# Autodesk Inventor assembly: Custom Cover v0.3
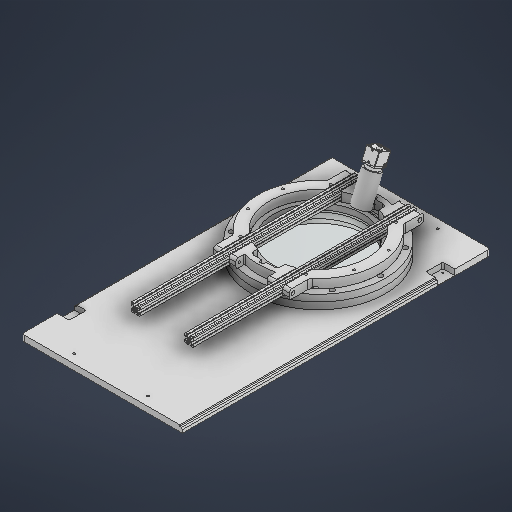
[picture p0: Inventor's stored thumbnail of the model, 512x512]
Saved by Autodesk Inventor 2025 (Build 290162000, 162)
## iProperties
Created: 2024-10-25
Part Number: Custom Cover v0.3
Document SubType Name: Assembly
Designer: mayhe
Author: mayhe
## Documents named in this file (15)
- C:\Users\mayhe\OneDrive\Documents\GitHub\In-situ-monitoring-of-powder-bed-fusion-additive-manufacturing\system_development\Orichalcum\v0.2\Hardware_design\custom-cover\Cover v 3\Custom Cover v0.3.iam
- C:\Users\mayhe\OneDrive\Documents\GitHub\In-situ-monitoring-of-powder-bed-fusion-additive-manufacturing\system_development\Orichalcum\v0.2\Hardware_design\custom-cover\cover\Updated Cover.ipt
- C:\Users\mayhe\OneDrive\Documents\GitHub\In-situ-monitoring-of-powder-bed-fusion-additive-manufacturing\system_development\Orichalcum\v0.2\Hardware_design\custom-cover\cylinder-parts\Cylinder 80-20 Spacer_2.ipt
- C:\Users\mayhe\OneDrive\Documents\GitHub\In-situ-monitoring-of-powder-bed-fusion-additive-manufacturing\system_development\Orichalcum\v0.2\Hardware_design\custom-cover\8020-parts\20-2020-500-CL.ipt
- C:\Users\mayhe\OneDrive\Documents\GitHub\In-situ-monitoring-of-powder-bed-fusion-additive-manufacturing\system_development\Orichalcum\v0.2\Hardware_design\custom-cover\cylinder-parts\Cylinder 80-20 Spacer_1 Slant.ipt
- C:\Users\mayhe\OneDrive\Documents\GitHub\In-situ-monitoring-of-powder-bed-fusion-additive-manufacturing\system_development\Orichalcum\v0.2\Hardware_design\Full Printer Assembly\Printer Body v6.ipt
- C:\Users\mayhe\OneDrive\Documents\GitHub\In-situ-monitoring-of-powder-bed-fusion-additive-manufacturing\system_development\Orichalcum\v0.2\Hardware_design\custom-cover\cylinder-parts\final-parts\Cylinder Bottom Ring.ipt
- C:\Users\mayhe\OneDrive\Documents\GitHub\In-situ-monitoring-of-powder-bed-fusion-additive-manufacturing\system_development\Orichalcum\v0.2\Hardware_design\custom-cover\cylinder-parts\Cylinder 80-20 Spacer_2 cable hole.ipt
- C:\Users\mayhe\OneDrive\Documents\GitHub\In-situ-monitoring-of-powder-bed-fusion-additive-manufacturing\system_development\Orichalcum\v0.2\Hardware_design\custom-cover\cylinder-parts\final-parts\Cylinder Slidey Bit Housing Camera + galvo.ipt
- C:\Users\mayhe\OneDrive\Documents\GitHub\In-situ-monitoring-of-powder-bed-fusion-additive-manufacturing\system_development\Orichalcum\v0.2\Hardware_design\custom-cover\cylinder-parts\cylinder-segments\Cylinder Segment  Camera + Galvo.ipt
- C:\Users\mayhe\OneDrive\Documents\GitHub\In-situ-monitoring-of-powder-bed-fusion-additive-manufacturing\system_development\Orichalcum\v0.2\Hardware_design\optical-camera\flircamera+lens.ipt
- C:\Users\mayhe\OneDrive\Documents\GitHub\In-situ-monitoring-of-powder-bed-fusion-additive-manufacturing\system_development\Orichalcum\v0.2\Hardware_design\pzt-parts\Substrate plates\substrate plate.ipt
- C:\Users\mayhe\OneDrive\Documents\GitHub\In-situ-monitoring-of-powder-bed-fusion-additive-manufacturing\system_development\Orichalcum\v0.2\Hardware_design\custom-cover\Cover v 3\260mm Housing 1.ipt
- C:\Users\mayhe\OneDrive\Documents\GitHub\In-situ-monitoring-of-powder-bed-fusion-additive-manufacturing\system_development\Orichalcum\v0.2\Hardware_design\custom-cover\Cover v 3\260 mm Glass.ipt
- C:\Users\mayhe\OneDrive\Documents\GitHub\In-situ-monitoring-of-powder-bed-fusion-additive-manufacturing\system_development\Orichalcum\v0.2\Hardware_design\custom-cover\Cover v 3\260mm housing 2.ipt
## Components (16 placed, 14 different names)
1. Printer Body v6:1 — Mate:49, Mate:50, Mate:51, Rotational:15
2. substrate plate:2 — Rotational:15
3. flircamera+lens:1 — Rotational:14
4. Cylinder Segment  Camera + Galvo:1 — Rotational:12, Mate:59, Rotational:13, Mate:60
5. Cylinder Slidey Bit Housing Camera + galvo:1 — Rotational:13, Mate:60, Rotational:14
6. Updated Cover:1 — Mate:49, Mate:50, Mate:51, Rotational:8
7. Cylinder Bottom Ring:1 — Rotational:8, Rotational:10, Rotational:11, Mate:52, Mate:54, Mate:56, Mate:58, Rotational:16
8. Cylinder 80-20 Spacer_1 Slant:2 — Rotational:16
9. Cylinder 80-20 Spacer_2 cable hole:1 — Rotational:11
10. Cylinder 80-20 Spacer_2:1 — Rotational:10, Rotational:12, Mate:59, Rotational:19
11. Cylinder 80-20 Spacer_1 Slant:1 — Mate:56, Mate:57, Mate:58
12. 20-2020-500-CL:1 — Mate:52
13. 20-2020-500-CL:2 — Mate:54, Mate:57
14. 260mm Housing 1:1 — Rotational:17, Rotational:18, Mate:61
15. 260 mm Glass:1 — Rotational:17
16. 260mm housing 2:1 — Rotational:18, Mate:61, Rotational:19
## Relationships (22: Mate 11, RevoluteJoint 11)
- Mate:49: Printer Body v6:1 ↔ Updated Cover:1
- Mate:50: Printer Body v6:1 ↔ Updated Cover:1
- Mate:51: Printer Body v6:1 ↔ Updated Cover:1
- Rotational:8 [RevoluteJoint]: Updated Cover:1 ↔ Cylinder Bottom Ring:1
- Rotational:10 [RevoluteJoint]: Cylinder Bottom Ring:1 ↔ Cylinder 80-20 Spacer_2:1
- Rotational:11 [RevoluteJoint]: Cylinder Bottom Ring:1 ↔ Cylinder 80-20 Spacer_2 cable hole:1
- Mate:52: Cylinder Bottom Ring:1 ↔ 20-2020-500-CL:1
- Mate:54: Cylinder Bottom Ring:1 ↔ 20-2020-500-CL:2
- Mate:56: Cylinder Bottom Ring:1 ↔ Cylinder 80-20 Spacer_1 Slant:1
- Mate:57: Cylinder 80-20 Spacer_1 Slant:1 ↔ 20-2020-500-CL:2
- Mate:58: Cylinder Bottom Ring:1 ↔ Cylinder 80-20 Spacer_1 Slant:1
- Rotational:12 [RevoluteJoint]: Cylinder Segment  Camera + Galvo:1 ↔ Cylinder 80-20 Spacer_2:1
- Mate:59: Cylinder Segment  Camera + Galvo:1 ↔ Cylinder 80-20 Spacer_2:1
- Rotational:13 [RevoluteJoint]: Cylinder Segment  Camera + Galvo:1 ↔ Cylinder Slidey Bit Housing Camera + galvo:1
- Mate:60: Cylinder Segment  Camera + Galvo:1 ↔ Cylinder Slidey Bit Housing Camera + galvo:1
- Rotational:14 [RevoluteJoint]: flircamera+lens:1 ↔ Cylinder Slidey Bit Housing Camera + galvo:1
- Rotational:15 [RevoluteJoint]: Printer Body v6:1 ↔ substrate plate:2
- Rotational:16 [RevoluteJoint]: Cylinder Bottom Ring:1 ↔ Cylinder 80-20 Spacer_1 Slant:2
- Rotational:17 [RevoluteJoint]: 260mm Housing 1:1 ↔ 260 mm Glass:1
- Rotational:18 [RevoluteJoint]: 260mm Housing 1:1 ↔ 260mm housing 2:1
- Mate:61: 260mm Housing 1:1 ↔ 260mm housing 2:1
- Rotational:19 [RevoluteJoint]: Cylinder 80-20 Spacer_2:1 ↔ 260mm housing 2:1
